# Autodesk Inventor assembly: EBF_900.1-top_w_cups
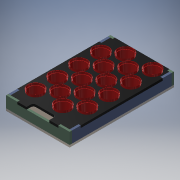
[picture p0: Inventor's stored thumbnail of the model, 180x180]
Saved by Autodesk Inventor 2019 (Build 230136000, 136)
## iProperties
Created: 2019-02-28
Part Number: EBF_900.1-top_w_cups
Document SubType Name: Assembly
Designer: Rene
Author: Rene
## Documents named in this file (7)
- C:\dev\c-scape\hardponics\dwg\eb_flow\EBF_900.1-water-tray_with_cups.iam
- C:\dev\c-scape\hardponics\dwg\eb_flow\EBF_001.1-top-plate_cup-holder.ipt
- C:\dev\c-scape\hardponics\dwg\eb_flow\XGEN_sambal-bakje.ipt
- C:\dev\c-scape\hardponics\dwg\eb_flow\EBF_002.1-side-plate_cup-holder.ipt
- C:\dev\c-scape\hardponics\dwg\eb_flow\EBF_003.1-front-plate_cup-holder.ipt
- C:\dev\c-scape\hardponics\dwg\eb_flow\EBF_004.1-back-plate_cup-holder.ipt
- C:\dev\c-scape\hardponics\dwg\eb_flow\EBF_005.1-bottom-plate_cup-holder.ipt
## Components (22 placed, 6 different names)
1. EBF_001.1-top-plate_cup-holder:1 — Mate:1, Mate:2, Mate:3, Mate:4, Mate:5, Flush:1, Mate:7, Flush:3, Flush:4, Mate:10, Flush:5, Flush:6
2. EBF_002.1-side-plate_cup-holder:1 — Mate:5, Flush:1, Mate:8, Flush:10
3. EBF_002.1-side-plate_cup-holder:2 — Mate:11, Flush:9, Mate:13
4. EBF_003.1-front-plate_cup-holder:1 — Mate:7, Flush:3, Flush:4, Mate:8, Mate:13
5. EBF_004.1-back-plate_cup-holder:1 — Mate:10, Flush:5, Flush:6, Flush:8, Mate:12
6. EBF_005.1-bottom-plate_cup-holder:1 — Flush:8, Mate:11, Flush:9, Flush:10, Mate:12
7. XGEN_sambal-bakje:1 — Mate:1, Mate:2
8. XGEN_sambal-bakje:2 — Mate:3, Mate:4
9. XGEN_sambal-bakje:3
10. XGEN_sambal-bakje:4
11. XGEN_sambal-bakje:5
12. XGEN_sambal-bakje:6
13. XGEN_sambal-bakje:7
14. XGEN_sambal-bakje:8
15. XGEN_sambal-bakje:9
16. XGEN_sambal-bakje:10
17. XGEN_sambal-bakje:11
18. XGEN_sambal-bakje:12
19. XGEN_sambal-bakje:13
20. XGEN_sambal-bakje:14
21. XGEN_sambal-bakje:15
22. XGEN_sambal-bakje:16
## Component patterns: (8 elements, first: XGEN_sambal-bakje:1 + XGEN_sambal-bakje:2)
## Relationships (19: Mate 11, Flush 8)
- Mate:1: EBF_001.1-top-plate_cup-holder:1 ↔ XGEN_sambal-bakje:1
- Mate:2: EBF_001.1-top-plate_cup-holder:1 ↔ XGEN_sambal-bakje:1
- Mate:3: EBF_001.1-top-plate_cup-holder:1 ↔ XGEN_sambal-bakje:2
- Mate:4: EBF_001.1-top-plate_cup-holder:1 ↔ XGEN_sambal-bakje:2
- Mate:5: EBF_001.1-top-plate_cup-holder:1 ↔ EBF_002.1-side-plate_cup-holder:1
- Flush:1: EBF_001.1-top-plate_cup-holder:1 ↔ EBF_002.1-side-plate_cup-holder:1
- Mate:7: EBF_001.1-top-plate_cup-holder:1 ↔ EBF_003.1-front-plate_cup-holder:1
- Flush:3: EBF_001.1-top-plate_cup-holder:1 ↔ EBF_003.1-front-plate_cup-holder:1
- Flush:4: EBF_001.1-top-plate_cup-holder:1 ↔ EBF_003.1-front-plate_cup-holder:1
- Mate:8: EBF_002.1-side-plate_cup-holder:1 ↔ EBF_003.1-front-plate_cup-holder:1
- Mate:10: EBF_001.1-top-plate_cup-holder:1 ↔ EBF_004.1-back-plate_cup-holder:1
- Flush:5: EBF_001.1-top-plate_cup-holder:1 ↔ EBF_004.1-back-plate_cup-holder:1
- Flush:6: EBF_001.1-top-plate_cup-holder:1 ↔ EBF_004.1-back-plate_cup-holder:1
- Flush:8: EBF_004.1-back-plate_cup-holder:1 ↔ EBF_005.1-bottom-plate_cup-holder:1
- Mate:11: EBF_002.1-side-plate_cup-holder:2 ↔ EBF_005.1-bottom-plate_cup-holder:1
- Flush:9: EBF_002.1-side-plate_cup-holder:2 ↔ EBF_005.1-bottom-plate_cup-holder:1
- Flush:10: EBF_002.1-side-plate_cup-holder:1 ↔ EBF_005.1-bottom-plate_cup-holder:1
- Mate:12: EBF_004.1-back-plate_cup-holder:1 ↔ EBF_005.1-bottom-plate_cup-holder:1
- Mate:13: EBF_002.1-side-plate_cup-holder:2 ↔ EBF_003.1-front-plate_cup-holder:1
